# Autodesk Inventor assembly: saponSEX_ver3
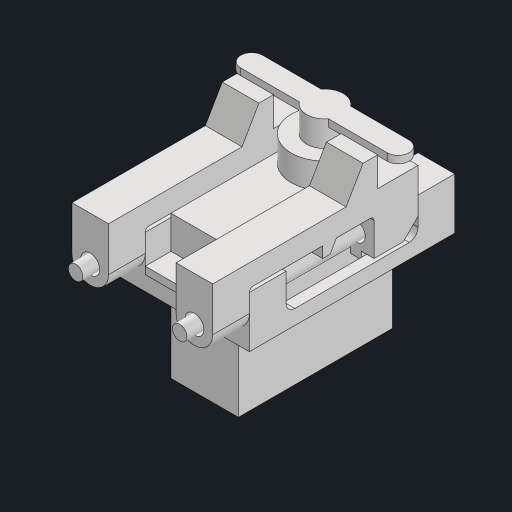
[picture p0: Inventor's stored thumbnail of the model, 512x512]
Saved by Autodesk Inventor 2023 (Build 270158000, 158)
## iProperties
Created: 2022-06-07
Part Number: saponSEX_ver3
Document SubType Name: Assembly
Designer: legot
Author: legot
## Documents named in this file (6)
- C:\Users\legot\OneDrive\ドキュメント\Inventor\HIKOSAPO\DropMechanism\saponSEX_ver3.iam
- C:\Users\legot\OneDrive\ドキュメント\Inventor\HIKOSAPO\DropMechanism\saponSEX_1.ipt
- C:\Users\legot\OneDrive\ドキュメント\Inventor\HIKOSAPO\public_parts\motor.ipt
- C:\Users\legot\OneDrive\ドキュメント\Inventor\HIKOSAPO\shaft2.ipt
- C:\Users\legot\OneDrive\ドキュメント\Inventor\HIKOSAPO\ナックル.ipt
- C:\Users\legot\OneDrive\ドキュメント\Inventor\HIKOSAPO\DropMechanism\saponSEX_2.ipt
## Components (7 placed, 5 different names)
1. saponSEX_1:1 — 挿入:4, 挿入:5, 挿入:8, メイト:1, メイト:2, メイト:3, 挿入:9
2. motor:1 — 挿入:3, 角度:1, 角度:2, メイト:1, メイト:2, メイト:3
3. shaft2:1 — 挿入:5
4. shaft2:2 — 挿入:4
5. ナックル:1 — 挿入:3
6. saponSEX_2:1 — 角度:2, 挿入:8
7. saponSEX_2:2 — 角度:1, 挿入:9
## Relationships (10: Insert 5, Mate 3, Angle 2)
- 挿入:3 [Insert]: motor:1 ↔ ナックル:1
- 挿入:4 [Insert]: saponSEX_1:1 ↔ shaft2:2
- 挿入:5 [Insert]: saponSEX_1:1 ↔ shaft2:1
- 角度:1 [Angle] (0 deg): motor:1 ↔ saponSEX_2:2
- 角度:2 [Angle] (0 deg): motor:1 ↔ saponSEX_2:1
- 挿入:8 [Insert]: saponSEX_1:1 ↔ saponSEX_2:1
- メイト:1 [Mate]: saponSEX_1:1 ↔ motor:1
- メイト:2 [Mate]: saponSEX_1:1 ↔ motor:1
- メイト:3 [Mate]: saponSEX_1:1 ↔ motor:1
- 挿入:9 [Insert]: saponSEX_1:1 ↔ saponSEX_2:2
